# Autodesk Inventor assembly: combined_mounts_v1
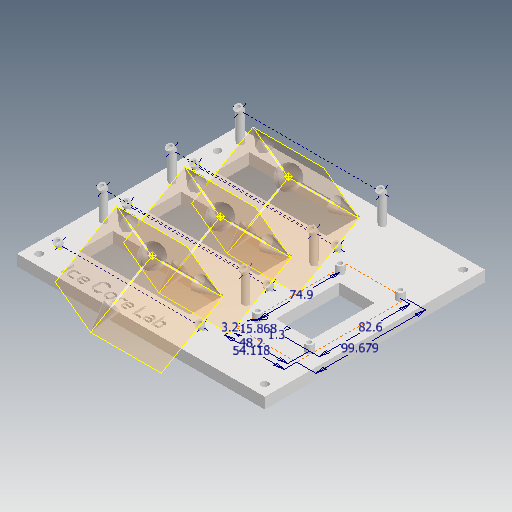
[picture p0: Inventor's stored thumbnail of the model, 512x512]
Saved by Autodesk Inventor 2025.1 (Build 291241000, 241)
## iProperties
Created: 2026-06-20
Part Number: combined_mounts_v1
Document SubType Name: Assembly
Designer: Aiden
Author: Aiden
## Documents named in this file (4)
- C:\Users\Aiden\Documents\GitHub\coldex-instrumentation\hardware\mounting_hardware\combined_mounts_v1.iam
- C:\Users\Aiden\Documents\GitHub\coldex-instrumentation\hardware\mounting_hardware\base_plate.ipt
- C:\Users\Aiden\Documents\GitHub\coldex-instrumentation\hardware\mounting_hardware\arduino_mega_standoffs.ipt
- C:\Users\Aiden\Documents\GitHub\coldex-instrumentation\hardware\mounting_hardware\relay_module_standoffs_angled.ipt
## Components (5 placed, 3 different names)
1. base_plate:1 — Mate:2, Mate:5
2. arduino_mega_standoffs:1 — Mate:5
3. relay_module_standoffs_angled:1 — Mate:2
4. relay_module_standoffs_angled:2
5. relay_module_standoffs_angled:3
## Component patterns: (3 elements, first: relay_module_standoffs_angled:1)
## Relationships (2: Mate 2)
- Mate:2: base_plate:1 ↔ relay_module_standoffs_angled:1
- Mate:5: base_plate:1 ↔ arduino_mega_standoffs:1
